# Autodesk Inventor assembly: 三組合窗頂
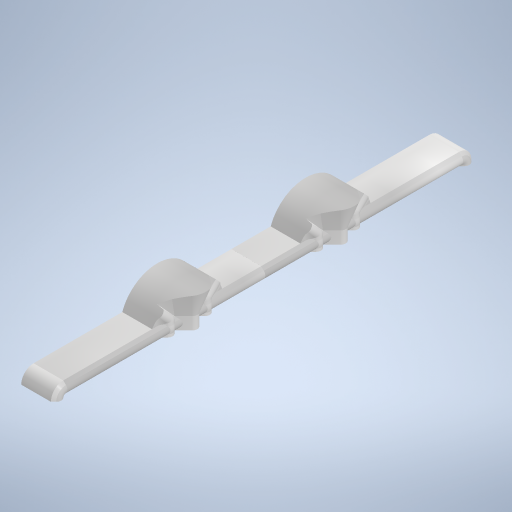
[picture p0: Inventor's stored thumbnail of the model, 512x512]
Saved by Autodesk Inventor 2024.2 (Build 282272000, 272)
## iProperties
Created: 2024-06-04
Part Number: 三組合窗頂
Document SubType Name: Assembly
Designer: User
Author: User
## Documents named in this file (3)
- C:\Users\User\OneDrive - 國立中山大學\桌面\創客基礎\final_project\三組合窗頂.iam
- C:\Users\User\OneDrive - 國立中山大學\桌面\創客基礎\final_project\三窗頂_1.ipt
- C:\Users\User\OneDrive - 國立中山大學\桌面\創客基礎\final_project\三窗頂_2.ipt
## Components (2 placed, 2 different names)
1. 三窗頂_1:1 — 貼合:1, 齊平:1, 齊平:2
2. 三窗頂_2:1 — 貼合:1, 齊平:1, 齊平:2
## Relationships (3: Flush 2, Mate 1)
- 貼合:1 [Mate]: 三窗頂_1:1 ↔ 三窗頂_2:1
- 齊平:1 [Flush]: 三窗頂_1:1 ↔ 三窗頂_2:1
- 齊平:2 [Flush]: 三窗頂_1:1 ↔ 三窗頂_2:1
